# Autodesk Inventor assembly: printer_larger
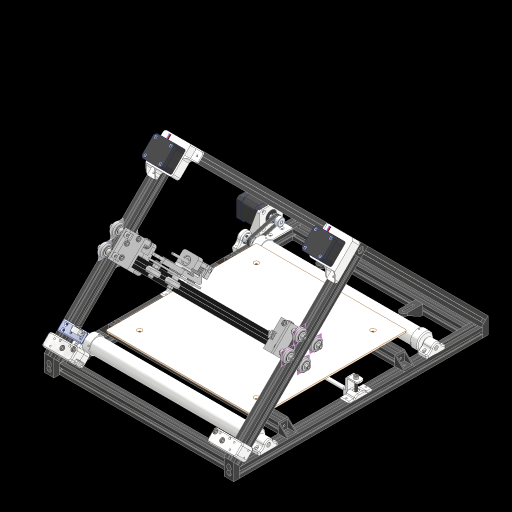
[picture p0: Inventor's stored thumbnail of the model, 512x512]
Saved by Autodesk Inventor 2023 (Build 270158000, 158)
## iProperties
Created: 2021-08-14
Part Number: printer_larger
Description: STEP AP214
Document SubType Name: Assembly
Designer: tandu
Sending System: SolidWorks 2020
Preprocessor: SwSTEP 2.0
Title: printer_larger.STEP
Revision Number: ANY
## Documents named in this file (38)
- C:\Users\tandu\Documents\GrabCAD\Custom Conveyor Belt 3D Printer\V1\Assembly\printer_largeeeprinter_larger.iam
- C:\Users\tandu\Documents\GrabCAD\Custom Conveyor Belt 3D Printer\V1\Assembly\printer_largeeeFrame.iam
- C:\Users\tandu\Documents\GrabCAD\Custom Conveyor Belt 3D Printer\V1\Assembly\printer_largeeeNEMA17_17HS19-2004S1_Stepperonline___ _________.ipt
- C:\Users\tandu\Documents\GrabCAD\Custom Conveyor Belt 3D Printer\V1\Assembly\printer_largeeetensioner_mount.ipt
- C:\Users\tandu\Documents\GrabCAD\Custom Conveyor Belt 3D Printer\V1\Assembly\printer_largeee5mm_roller_shaft.ipt
- C:\Users\tandu\Documents\GrabCAD\Custom Conveyor Belt 3D Printer\V1\Assembly\printer_largeee330mm_cf_tube_thin.ipt
- C:\Users\tandu\Documents\GrabCAD\Custom Conveyor Belt 3D Printer\V1\Assembly\printer_largeee605_bearing.ipt
- C:\Users\tandu\Documents\GrabCAD\Custom Conveyor Belt 3D Printer\V1\Assembly\printer_largeeetube_mount_motor_side.ipt
- C:\Users\tandu\Documents\GrabCAD\Custom Conveyor Belt 3D Printer\V1\Assembly\printer_largeeeGT2_20T_____________1.ipt
- C:\Users\tandu\Documents\GrabCAD\Custom Conveyor Belt 3D Printer\V1\Assembly\printer_largeeeflange_coupling.ipt
- C:\Users\tandu\Documents\GrabCAD\Custom Conveyor Belt 3D Printer\V1\Assembly\printer_largeeetube_holder_motor_side.ipt
- C:\Users\tandu\Documents\GrabCAD\Custom Conveyor Belt 3D Printer\V1\Assembly\printer_largeeebelt_motor_mount.ipt
- C:\Users\tandu\Documents\GrabCAD\Custom Conveyor Belt 3D Printer\V1\Assembly\printer_largeeebed_mount_300mm.ipt
- C:\Users\tandu\Documents\GrabCAD\Custom Conveyor Belt 3D Printer\V1\Assembly\printer_largeee330mm_cf_tube.ipt
- C:\Users\tandu\Documents\GrabCAD\Custom Conveyor Belt 3D Printer\V1\Assembly\printer_largeeebed_mount_bracket.ipt
- C:\Users\tandu\Documents\GrabCAD\Custom Conveyor Belt 3D Printer\V1\Assembly\printer_largeeetube_holder.ipt
- C:\Users\tandu\Documents\GrabCAD\Custom Conveyor Belt 3D Printer\V1\Assembly\printer_largeeetube_mount.ipt
- C:\Users\tandu\Documents\GrabCAD\Custom Conveyor Belt 3D Printer\V1\Assembly\printer_largeeeroller_rod.ipt
- C:\Users\tandu\Documents\GrabCAD\Custom Conveyor Belt 3D Printer\V1\Assembly\printer_largeeeramp_mount.ipt
- C:\Users\tandu\Documents\GrabCAD\Custom Conveyor Belt 3D Printer\V1\Assembly\printer_largeeebed_Predeterminado.ipt
- C:\Users\tandu\Documents\GrabCAD\Custom Conveyor Belt 3D Printer\V1\Assembly\printer_largeeeBelt2-2987^printer_larger.ipt
- C:\Users\tandu\Documents\GrabCAD\Custom Conveyor Belt 3D Printer\V1\Assembly\printer_largeeeF695 Bearing.step.ipt
- C:\Users\tandu\Documents\GrabCAD\Custom Conveyor Belt 3D Printer\V1\Assembly\printer_largeeeleft_motor_mount.ipt
- C:\Users\tandu\Documents\GrabCAD\Custom Conveyor Belt 3D Printer\V1\Assembly\printer_largeeeM5x40.ipt
- C:\Users\tandu\Documents\GrabCAD\Custom Conveyor Belt 3D Printer\V1\Assembly\printer_largeeeright_motor_mount.ipt
- C:\Users\tandu\Documents\GrabCAD\Custom Conveyor Belt 3D Printer\V1\Assembly\printer_largeeegantry_idler_left.ipt
- C:\Users\tandu\Documents\GrabCAD\Custom Conveyor Belt 3D Printer\V1\Assembly\printer_largeeegantry_idler_right.ipt
- C:\Users\tandu\Documents\GrabCAD\Custom Conveyor Belt 3D Printer\V1\Assembly\printer_largeeegantry_idler_left_top.ipt
- C:\Users\tandu\Documents\GrabCAD\Custom Conveyor Belt 3D Printer\V1\Assembly\printer_largeeegantry_idler_right_top.ipt
- C:\Users\tandu\Documents\GrabCAD\Custom Conveyor Belt 3D Printer\V1\Assembly\printer_largeeetensioner_mount_mount.ipt
- C:\Users\tandu\Documents\GrabCAD\Custom Conveyor Belt 3D Printer\V1\Assembly\printer_largeeeM5x30.ipt
- C:\Users\tandu\Documents\GrabCAD\Custom Conveyor Belt 3D Printer\V1\Assembly\printer_largeeey_switch_mount.ipt
- C:\Users\tandu\Documents\GrabCAD\Custom Conveyor Belt 3D Printer\V1\Assembly\printer_largeeelimit_switch_cover_y.ipt
- C:\Users\tandu\Documents\GrabCAD\Custom Conveyor Belt 3D Printer\V1\Assembly\printer_largeeeMicroswitch2.step_1.iam
- C:\Users\tandu\Documents\GrabCAD\Custom Conveyor Belt 3D Printer\V1\Assembly\printer_largeeebearing_spacer.ipt
- C:\Users\tandu\Documents\GrabCAD\Custom Conveyor Belt 3D Printer\References\Roller based conveyor belt 3d printer\LeftGantryMount.iam
- C:\Users\tandu\Documents\GrabCAD\Custom Conveyor Belt 3D Printer\References\Roller based conveyor belt 3d printer\RightGantryMount.iam
- C:\Users\tandu\Documents\GrabCAD\Custom Conveyor Belt 3D Printer\References\Roller based conveyor belt 3d printer\RollerVersionExtruder.iam
## Components (70 placed, 70 different names)
1. Frame_1 [sub-assembly] — Tangent:1, Mate:7, Angle:1, Symmetry:1, Tangent:2
2. ramp_mount_34
3. ramp_mount_35
4. bearing_spacer_96
5. bearing_spacer_95
6. F695 Bearing.step_44
7. F695 Bearing.step_45
8. gantry_idler_left_59
9. gantry_idler_right_60
10. F695 Bearing.step_61
11. F695 Bearing.step_62
12. F695 Bearing.step_63
13. F695 Bearing.step_64
14. F695 Bearing.step_65
15. F695 Bearing.step_66
16. gantry_idler_left_top_71
17. gantry_idler_right_top_72
18. M5x40_76
19. M5x40_80
20. M5x40_81
21. M5x40_82
22. LeftGantryMount:1 [sub-assembly] — Tangent:1, Mate:8, Tangent:2, Mate:9, Mate:10, Mate:11
23. RightGantryMount:1 [sub-assembly] — Mate:12, Mate:13, Mate:14
24. RollerVersionExtruder:1 [sub-assembly] — Mate:9, Mate:10, Mate:11, Mate:12, Mate:13, Mate:14
25. y_switch_mount_91
26. limit_switch_cover_y_92
27. Microswitch2.step_93 [sub-assembly]
28. flange_coupling_14
29. 5mm_roller_shaft_13
30. 605_bearing_9
31. GT2_20T_____________1_11
32. 5mm_roller_shaft_5
33. 5mm_roller_shaft_6
34. roller_rod_33
35. roller_rod_30
36. roller_rod_28
37. tube_holder_25
38. bed_Predeterminado_36
39. tensioner_mount_4
40. tensioner_mount_7
41. 330mm_cf_tube_thin_8
42. tube_mount_motor_side_10
43. tube_holder_motor_side_15
44. 330mm_cf_tube_19
45. 330mm_cf_tube_20
46. tube_holder_26
47. tube_mount_27
48. tube_mount_29
49. tube_holder_31
50. tube_mount_32
51. tensioner_mount_mount_85
52. M5x30_86
53. tensioner_mount_mount_87
54. M5x30_88
55. NEMA17_17HS19-2004S1_Stepperonline___ __________2
56. NEMA17_17HS19-2004S1_Stepperonline___ __________39
57. NEMA17_17HS19-2004S1_Stepperonline___ __________40
58. belt_motor_mount_16
59. left_motor_mount_53
60. right_motor_mount_58
61. GT2_20T_____________1_12
62. Belt2-2987^printer_larger_38
63. GT2_20T_____________1_41
64. GT2_20T_____________1_42
65. bed_mount_300mm_17
66. bed_mount_300mm_18
67. bed_mount_bracket_21
68. bed_mount_bracket_22
69. bed_mount_bracket_23
70. bed_mount_bracket_24
## Relationships (12: Mate 8, Tangent 2, Angle 1, Symmetry 1)
- Tangent:1: Frame_1 ↔ LeftGantryMount:1
- Mate:7: Frame_1
- Angle:1 (0 deg): Frame_1
- Symmetry:1: Frame_1
- Mate:8: LeftGantryMount:1
- Tangent:2: Frame_1 ↔ LeftGantryMount:1
- Mate:9: LeftGantryMount:1 ↔ RollerVersionExtruder:1
- Mate:10: LeftGantryMount:1 ↔ RollerVersionExtruder:1
- Mate:11: LeftGantryMount:1 ↔ RollerVersionExtruder:1
- Mate:12: RightGantryMount:1 ↔ RollerVersionExtruder:1
- Mate:13: RightGantryMount:1 ↔ RollerVersionExtruder:1
- Mate:14: RightGantryMount:1 ↔ RollerVersionExtruder:1
